# Autodesk Inventor assembly: MK3 Master Structure
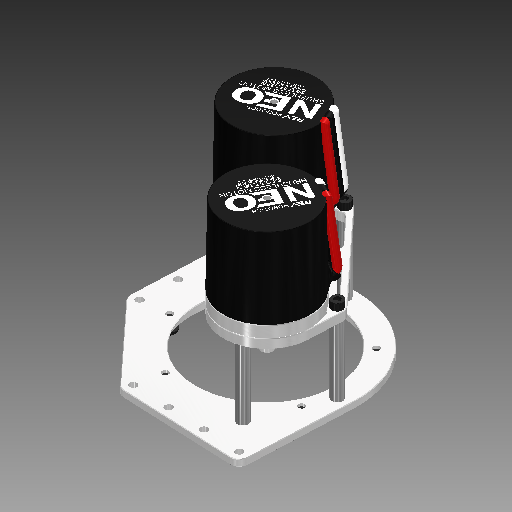
[picture p0: Inventor's stored thumbnail of the model, 512x512]
Saved by Autodesk Inventor 2025 (Build 290162010, 162A)
## iProperties
Created: 2024-07-31
Part Number: MK3 Master Structure
Document SubType Name: Assembly
Designer: rohan
Author: rohan
## Documents named in this file (18)
- D:\ultimate-hecker\Computer-Aided-Design\FRC-Offseason-Design-Training\Parts Library\Drivetrains\Swerve Modules\MK3\MK3 Master Structure.iam
- D:\ultimate-hecker\Computer-Aided-Design\FRC-Offseason-Design-Training\Parts Library\Drivetrains\Swerve Modules\MK3\MK3 Motor Mounting Plate.ipt
- D:\ultimate-hecker\Computer-Aided-Design\FRC-Offseason-Design-Training\Parts Library\Drivetrains\Swerve Modules\MK3\MK3 Motor Spacers.ipt
- D:\ultimate-hecker\Computer-Aided-Design\FRC-Offseason-Design-Training\Parts Library\Drivetrains\Swerve Modules\MK3\MK3 Main Plate.ipt
- D:\ultimate-hecker\Computer-Aided-Design\FRC-Offseason-Design-Training\Parts Library\Hardware\Spacers\Spacers & Standoffs.ipt
- D:\ultimate-hecker\Computer-Aided-Design\FRC-Offseason-Design-Training\Parts Library\Hardware\Spacers\Spacers & Standoffs\Aluminum Unthreaded Spacer (No. 10 x 1.875Lg x 0.313OD).ipt
- D:\ultimate-hecker\Computer-Aided-Design\FRC-Offseason-Design-Training\Parts Library\Motors\FRC\NEO.ipt
- D:\ultimate-hecker\Computer-Aided-Design\FRC-Offseason-Design-Training\Parts Library\Hardware\Fasteners\Machine Screws\10-32 UNFx2.5 Socket Head Cap Screw.ipt
- D:\ultimate-hecker\Computer-Aided-Design\FRC-Offseason-Design-Training\Parts Library\Hardware\Fasteners\Machine Screws.ipt
- D:\ultimate-hecker\Computer-Aided-Design\FRC-Offseason-Design-Training\Parts Library\Hardware\Fasteners\Machine Screws\10-32 UNFx2.75 Socket Head Cap Screw.ipt
- D:\ultimate-hecker\Computer-Aided-Design\FRC-Offseason-Design-Training\Parts Library\Hardware\Fasteners\Machine Screws\10-32 UNFx0.625 Socket Head Cap Screw.ipt
- D:\ultimate-hecker\Computer-Aided-Design\FRC-Offseason-Design-Training\Parts Library\Electronics\FRC\Sensors\CTRE Mag Encoder.ipt
- D:\ultimate-hecker\Computer-Aided-Design\FRC-Offseason-Design-Training\Parts Library\Power Transfer\Bearings and Bushings\Bearings\F689-ZZ Bearing.ipt
- D:\ultimate-hecker\Computer-Aided-Design\FRC-Offseason-Design-Training\Parts Library\Drivetrains\Swerve Modules\MK2\MK2 Steering Shaft.iam
- D:\ultimate-hecker\Computer-Aided-Design\FRC-Offseason-Design-Training\Parts Library\Power Transfer\Bearings and Bushings\Bearings\R188ZZ Bearing.ipt
- D:\ultimate-hecker\Computer-Aided-Design\FRC-Offseason-Design-Training\Parts Library\Hardware\Fasteners\Machine Key, 2 X 2 X 12mm.ipt
- D:\ultimate-hecker\Computer-Aided-Design\FRC-Offseason-Design-Training\Parts Library\Hardware\Fasteners\Machine Screws\10-32 UNFx0.25 Button Head Cap Screw.ipt
- D:\ultimate-hecker\Computer-Aided-Design\FRC-Offseason-Design-Training\Parts Library\Hardware\Spacers\Spacers & Standoffs\SDS Neo Shaft Spacer 0.437.ipt
## Components (28 placed, 15 different names)
1. MK3 Motor Mounting Plate:1 — Insert:3, Insert:4, Insert:7, Insert:8, Insert:9, Insert:10, Insert:11, Insert:12, Insert:19, Insert:20, Insert:21, Insert:22, Insert:23
2. MK3 Motor Spacers:1 — Insert:7, Insert:8, Insert:15, Insert:16
3. MK3 Motor Spacers:2 — Insert:9, Insert:10, Insert:17, Insert:18
4. MK3 Main Plate:1 — Insert:1, Insert:2, Insert:5, Insert:6, Insert:13, Insert:14, Insert:24, Insert:27, Insert:28, Insert:29, Insert:30, Insert:31
5. Aluminum Unthreaded Spacer (No. 10 x 1.875Lg x 0.313OD):1 — Insert:6
6. Aluminum Unthreaded Spacer (No. 10 x 1.875Lg x 0.313OD):2 — Insert:5
7. Aluminum Unthreaded Spacer (No. 10 x 1.875Lg x 0.313OD):3 — Insert:2, Insert:4
8. Aluminum Unthreaded Spacer (No. 10 x 1.875Lg x 0.313OD):4 — Insert:1, Insert:3
9. NEO:1 — Insert:15, Insert:16, Insert:32, Mate:1, Insert:34
10. NEO:2 — Insert:17, Insert:18, Insert:33
11. 10-32 UNFx2.5 Socket Head Cap Screw:1 — Insert:11
12. 10-32 UNFx2.5 Socket Head Cap Screw:2 — Insert:12
13. 10-32 UNFx2.75 Socket Head Cap Screw:3 — Insert:13
14. 10-32 UNFx2.75 Socket Head Cap Screw:4 — Insert:14
15. 10-32 UNFx0.625 Socket Head Cap Screw:5 — Insert:19
16. 10-32 UNFx0.625 Socket Head Cap Screw:6 — Insert:20
17. CTRE Mag Encoder:1 — Insert:21, Insert:22
18. F689-ZZ Bearing:1 — Insert:23
19. MK2 Steering Shaft:1 [sub-assembly] — Insert:25
20. R188ZZ Bearing:1 — Insert:24, Insert:25
21. 10-32 UNFx0.25 Button Head Cap Screw:7 — Insert:29
22. 10-32 UNFx0.25 Button Head Cap Screw:8 — Insert:28
23. 10-32 UNFx0.25 Button Head Cap Screw:9 — Insert:27
24. 10-32 UNFx0.25 Button Head Cap Screw:10 — Insert:30
25. 10-32 UNFx0.25 Button Head Cap Screw:11 — Insert:31
26. Machine Key, 2 X 2 X 12mm:2 — Insert:32, Mate:1
27. SDS Neo Shaft Spacer 0.437:5 — Insert:33
28. SDS Neo Shaft Spacer 0.437:6 — Insert:34
## Relationships (34: Insert 33, Mate 1)
- Insert:1: MK3 Main Plate:1 ↔ Aluminum Unthreaded Spacer (No. 10 x 1.875Lg x 0.313OD):4
- Insert:2: MK3 Main Plate:1 ↔ Aluminum Unthreaded Spacer (No. 10 x 1.875Lg x 0.313OD):3
- Insert:3: MK3 Motor Mounting Plate:1 ↔ Aluminum Unthreaded Spacer (No. 10 x 1.875Lg x 0.313OD):4
- Insert:4: MK3 Motor Mounting Plate:1 ↔ Aluminum Unthreaded Spacer (No. 10 x 1.875Lg x 0.313OD):3
- Insert:5: MK3 Main Plate:1 ↔ Aluminum Unthreaded Spacer (No. 10 x 1.875Lg x 0.313OD):2
- Insert:6: MK3 Main Plate:1 ↔ Aluminum Unthreaded Spacer (No. 10 x 1.875Lg x 0.313OD):1
- Insert:7: MK3 Motor Mounting Plate:1 ↔ MK3 Motor Spacers:1
- Insert:8: MK3 Motor Mounting Plate:1 ↔ MK3 Motor Spacers:1
- Insert:9: MK3 Motor Mounting Plate:1 ↔ MK3 Motor Spacers:2
- Insert:10: MK3 Motor Mounting Plate:1 ↔ MK3 Motor Spacers:2
- Insert:11: MK3 Motor Mounting Plate:1 ↔ 10-32 UNFx2.5 Socket Head Cap Screw:1
- Insert:12: MK3 Motor Mounting Plate:1 ↔ 10-32 UNFx2.5 Socket Head Cap Screw:2
- Insert:13: MK3 Main Plate:1 ↔ 10-32 UNFx2.75 Socket Head Cap Screw:3
- Insert:14: MK3 Main Plate:1 ↔ 10-32 UNFx2.75 Socket Head Cap Screw:4
- Insert:15: MK3 Motor Spacers:1 ↔ NEO:1
- Insert:16: MK3 Motor Spacers:1 ↔ NEO:1
- Insert:17: MK3 Motor Spacers:2 ↔ NEO:2
- Insert:18: MK3 Motor Spacers:2 ↔ NEO:2
- Insert:19: MK3 Motor Mounting Plate:1 ↔ 10-32 UNFx0.625 Socket Head Cap Screw:5
- Insert:20: MK3 Motor Mounting Plate:1 ↔ 10-32 UNFx0.625 Socket Head Cap Screw:6
- Insert:21: MK3 Motor Mounting Plate:1 ↔ CTRE Mag Encoder:1
- Insert:22: MK3 Motor Mounting Plate:1 ↔ CTRE Mag Encoder:1
- Insert:23: MK3 Motor Mounting Plate:1 ↔ F689-ZZ Bearing:1
- Insert:24: MK3 Main Plate:1 ↔ R188ZZ Bearing:1
- Insert:25: MK2 Steering Shaft:1 ↔ R188ZZ Bearing:1
- Insert:27: MK3 Main Plate:1 ↔ 10-32 UNFx0.25 Button Head Cap Screw:9
- Insert:28: MK3 Main Plate:1 ↔ 10-32 UNFx0.25 Button Head Cap Screw:8
- Insert:29: MK3 Main Plate:1 ↔ 10-32 UNFx0.25 Button Head Cap Screw:7
- Insert:30: MK3 Main Plate:1 ↔ 10-32 UNFx0.25 Button Head Cap Screw:10
- Insert:31: MK3 Main Plate:1 ↔ 10-32 UNFx0.25 Button Head Cap Screw:11
- Insert:32: NEO:1 ↔ Machine Key, 2 X 2 X 12mm:2
- Mate:1: NEO:1 ↔ Machine Key, 2 X 2 X 12mm:2
- Insert:33: NEO:2 ↔ SDS Neo Shaft Spacer 0.437:5
- Insert:34: NEO:1 ↔ SDS Neo Shaft Spacer 0.437:6
